# Autodesk Inventor assembly: Whistle Mk 3.0
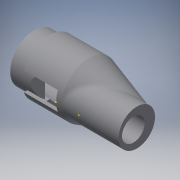
[picture p0: Inventor's stored thumbnail of the model, 180x180]
Saved by Autodesk Inventor 2019 (Build 230136000, 136)
## iProperties
Created: 2019-10-01
Part Number: Whistle Mk 3.0
Document SubType Name: Assembly
Designer: Kepler
Author: Kepler
## Documents named in this file (3)
- C:\Users\Kepler\Documents\Inventor\Whistles\Whistle Mk 3.0.iam
- C:\Users\Kepler\Documents\Inventor\Whistles\Whistle Exterior 3.0.ipt
- C:\Users\Kepler\Documents\Inventor\Whistles\Whistle 3.0.ipt
## Components (2 placed, 2 different names)
1. Whistle Exterior 3.0:1 — Mate:1
2. Whistle 3.0:1 — Mate:1
## Relationships (1: Mate 1)
- Mate:1: Whistle Exterior 3.0:1 ↔ Whistle 3.0:1
